# Autodesk Inventor assembly: assy-shooter_base
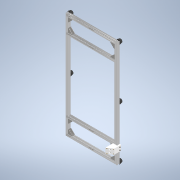
[picture p0: Inventor's stored thumbnail of the model, 180x180]
Saved by Autodesk Inventor 2022 (Build 260153000, 153)
## iProperties
Created: 2021-10-14
Part Number: assy-shooter_base
Document SubType Name: Assembly
Designer: yuto6
Author: yuto6
## Documents named in this file (3)
- C:\Users\yuto6\Documents\catchrobo_hardware\assy-shooter\assy-shooter_base.iam
- C:\Users\yuto6\Documents\catchrobo_hardware\assy-shooter\s-assy-shooter_frame.iam
- C:\Users\yuto6\Documents\catchrobo_hardware\assy-shooter\s-assy-frame-connector.iam
## Components (2 placed, 2 different names)
1. s-assy-shooter_frame:1 [sub-assembly] — メイト:1, メイト:2, フラッシュ:1
2. s-assy-frame-connector:1 [sub-assembly] — メイト:1, メイト:2, フラッシュ:1
## Relationships (3: Mate 2, Flush 1)
- メイト:1 [Mate]: s-assy-shooter_frame:1 ↔ s-assy-frame-connector:1
- メイト:2 [Mate]: s-assy-shooter_frame:1 ↔ s-assy-frame-connector:1
- フラッシュ:1 [Flush] (90 mm): s-assy-shooter_frame:1 ↔ s-assy-frame-connector:1
